# Autodesk Inventor assembly: ASY Рама №1 платформа
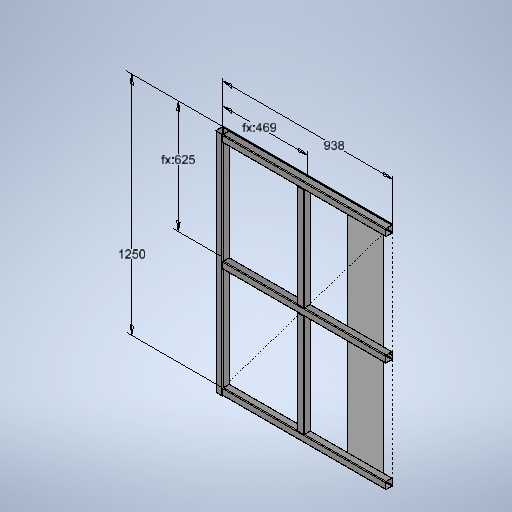
[picture p0: Inventor's stored thumbnail of the model, 512x512]
Saved by Autodesk Inventor 2025 (Build 290162010, 162A)
## iProperties
_SolveAssemblyDoc: Frame Generator Solve Assembly
_Version: 25.0.0
Created: 2025-01-19
Part Number: ASY Рама №1 платформа
Document SubType Name: Assembly
Designer: pokla
Author: pokla
## Documents named in this file (4)
- C:\Users\pokla\Documents\Inventor\NDM-VOS_powder_hopper\ASY Рама №1 платформа.iam
- C:\Users\pokla\Documents\Inventor\NDM-VOS_powder_hopper\ASY Рама №1 платформа.ipt
- C:\Users\pokla\Documents\Inventor\NDM-VOS_powder_hopper\ASY Рама №1 платформа\Frame\Frame 1737397310968.iam
- C:\Users\pokla\Documents\Inventor\NDM-VOS_powder_hopper\Ограждающий борт.ipt
## Components (3 placed, 3 different names)
1. ASY Рама №1 платформа:1
2. Frame 1737397310968:1 [sub-assembly] — Mate:1, Flush:1, Flush:2
3. Ограждающий борт:1 — Mate:1, Flush:1, Flush:2
## Relationships (3: Flush 2, Mate 1)
- Mate:1: Frame 1737397310968:1 ↔ Ограждающий борт:1
- Flush:1: Frame 1737397310968:1 ↔ Ограждающий борт:1
- Flush:2 (50 mm): Frame 1737397310968:1 ↔ Ограждающий борт:1
